# Autodesk Inventor assembly: Gearboxes_DesignTraining_Exercise1
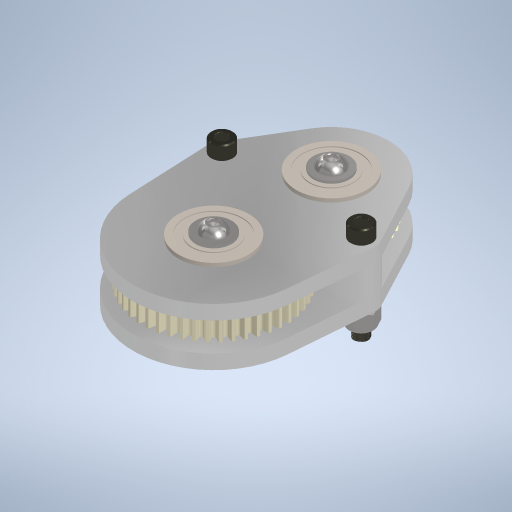
[picture p0: Inventor's stored thumbnail of the model, 512x512]
Saved by Autodesk Inventor 2024 (Build 280153000, 153)
## iProperties
Created: 2024-07-22
Part Number: Gearboxes_DesignTraining_Exercise1
Document SubType Name: Assembly
Designer: Danielle
Author: Danielle
## Documents named in this file (12)
- C:\Users\micha\OneDrive\Documents\GitHub\1622-2024-Assignments\Danielle\Gearboxes_DesignTraining_Exercise1.iam
- C:\Users\micha\OneDrive\Documents\BottomPlate.ipt
- C:\Users\micha\OneDrive\Documents\TopPlate.ipt
- C:\Users\micha\Downloads\WCP-0707 (1)\WCP-0707 (1).ipt
- C:\Users\micha\Downloads\WCP-0188 (1)\WCP-0188 (1).ipt
- C:\Users\micha\Downloads\WCP-0783 (1)\WCP-0783 (1).ipt
- C:\Users\micha\Downloads\WCP-0783\0.5 in long x 0.5 in wide x 0.257 in tap standoff.ipt
- C:\Users\micha\OneDrive\Documents\1.123 in. Hex Shaft.ipt
- C:\Users\micha\Downloads\92949A535_18-8 Stainless Steel Button Head Hex Drive Screw\92949A535_18-8 Stainless Steel Button Head Hex Drive Screw.ipt
- C:\Users\micha\Downloads\90107A029_316 Stainless Steel Washer\90107A029_316 Stainless Steel Washer.ipt
- C:\Users\micha\OneDrive\Documents\GitHub\1622-2024-Assignments\COTS Library\Fasteners\Bolts\Socket-Head\0.25-20\COTS_90044A123_Black-Oxide Alloy Steel Socket Head Screw.ipt
- C:\Users\micha\Downloads\97135A414_High-Strength Steel Nylon-Insert Locknut (1)\97135A414_High-Strength Steel Nylon-Insert Locknut (1).ipt
## Components (24 placed, 11 different names)
1. BottomPlate:1 — Mate:1, Mate:2, Mate:3, Mate:4, Mate:5, Mate:6, Mate:7, Mate:8, Mate:13, Mate:14, Mate:15, Mate:16, Mate:17, Mate:18, Mate:47, Mate:48
2. TopPlate:1 — Mate:1, Mate:2, Mate:3, Mate:4, Mate:9, Mate:10, Mate:11, Mate:12, Flush:5, Flush:6, Flush:7, Mate:41, Mate:42, Mate:43, Mate:44
3. WCP-0707 (1):1 — Mate:6, Flush:1, Flush:2, Angle:1, Angle:2
4. WCP-0188 (1):1 — Mate:5, Flush:1, Flush:2, Mate:19, Mate:20, Angle:3, Angle:4
5. WCP-0783 (1):1 — Mate:8, Mate:14, Angle:1, Mate:28
6. WCP-0783 (1):2 — Mate:10, Mate:11, Angle:2, Flush:9, Mate:22, Angle:5, Mate:26
7. WCP-0783 (1):3 — Mate:9, Mate:12, Mate:20, Angle:4, Mate:21, Flush:8, Angle:6, Mate:24
8. WCP-0783 (1):4 — Mate:7, Mate:13, Mate:19, Angle:3, Mate:29, Mate:30
9. 0.5 in long x 0.5 in wide x 0.257 in tap standoff:1 — Mate:15, Mate:16
10. 0.5 in long x 0.5 in wide x 0.257 in tap standoff:2 — Mate:17, Mate:18
11. 1.123 in. Hex Shaft:1 — Mate:21, Flush:8, Angle:6, Mate:23, Mate:31, Mate:33, Mate:35, Angle:8
12. 1.123 in. Hex Shaft:2 — Flush:9, Mate:22, Angle:5, Mate:25, Mate:27, Mate:32, Mate:34, Angle:7, Mate:36
13. 92949A535_18-8 Stainless Steel Button Head Hex Drive Screw:1 — Mate:33, Mate:39
14. 90107A029_316 Stainless Steel Washer:1 — Mate:23, Mate:24, Mate:35, Mate:39
15. 92949A535_18-8 Stainless Steel Button Head Hex Drive Screw:2 — Mate:32, Mate:37
16. 90107A029_316 Stainless Steel Washer:2 — Mate:29, Mate:30, Angle:8, Mate:38
17. 92949A535_18-8 Stainless Steel Button Head Hex Drive Screw:3 — Mate:31, Mate:38
18. 90107A029_316 Stainless Steel Washer:3 — Mate:25, Mate:26, Angle:7, Mate:40
19. 92949A535_18-8 Stainless Steel Button Head Hex Drive Screw:4 — Mate:34, Mate:40
20. 90107A029_316 Stainless Steel Washer:4 — Mate:27, Mate:28, Mate:36, Mate:37
21. COTS_90044A123_Black-Oxide Alloy Steel Socket Head Screw:1 — Mate:41, Mate:42, Mate:45
22. COTS_90044A123_Black-Oxide Alloy Steel Socket Head Screw:2 — Mate:43, Mate:44, Mate:46
23. 97135A414_High-Strength Steel Nylon-Insert Locknut (1):1 — Mate:45, Mate:47
24. 97135A414_High-Strength Steel Nylon-Insert Locknut (1):2 — Mate:46, Mate:48
## Relationships (63: Mate 48, Angle 8, Flush 7)
- Mate:1: BottomPlate:1 ↔ TopPlate:1
- Mate:2: BottomPlate:1 ↔ TopPlate:1
- Mate:3: BottomPlate:1 ↔ TopPlate:1
- Mate:4: BottomPlate:1 ↔ TopPlate:1
- Mate:5: BottomPlate:1 ↔ WCP-0188 (1):1
- Mate:6: BottomPlate:1 ↔ WCP-0707 (1):1
- Flush:1: WCP-0707 (1):1 ↔ WCP-0188 (1):1
- Mate:7: BottomPlate:1 ↔ WCP-0783 (1):4
- Mate:8: BottomPlate:1 ↔ WCP-0783 (1):1
- Mate:9: TopPlate:1 ↔ WCP-0783 (1):3
- Mate:10: TopPlate:1 ↔ WCP-0783 (1):2
- Mate:11: TopPlate:1 ↔ WCP-0783 (1):2
- Mate:12: TopPlate:1 ↔ WCP-0783 (1):3
- Mate:13: BottomPlate:1 ↔ WCP-0783 (1):4
- Mate:14: BottomPlate:1 ↔ WCP-0783 (1):1
- Mate:15: BottomPlate:1 ↔ 0.5 in long x 0.5 in wide x 0.257 in tap standoff:1
- Mate:16: BottomPlate:1 ↔ 0.5 in long x 0.5 in wide x 0.257 in tap standoff:1
- Mate:17: BottomPlate:1 ↔ 0.5 in long x 0.5 in wide x 0.257 in tap standoff:2
- Mate:18: BottomPlate:1 ↔ 0.5 in long x 0.5 in wide x 0.257 in tap standoff:2
- Flush:2: WCP-0707 (1):1 ↔ WCP-0188 (1):1
- Mate:19: WCP-0188 (1):1 ↔ WCP-0783 (1):4
- Mate:20: WCP-0188 (1):1 ↔ WCP-0783 (1):3
- Angle:1 (0 deg): WCP-0707 (1):1 ↔ WCP-0783 (1):1
- Angle:2 (0 deg): WCP-0707 (1):1 ↔ WCP-0783 (1):2
- Angle:3 (0 deg): WCP-0188 (1):1 ↔ WCP-0783 (1):4
- Angle:4 (0 deg): WCP-0188 (1):1 ↔ WCP-0783 (1):3
- Flush:5: TopPlate:1
- Flush:6: TopPlate:1
- Flush:7: TopPlate:1
- Mate:21: WCP-0783 (1):3 ↔ 1.123 in. Hex Shaft:1
- Flush:8: WCP-0783 (1):3 ↔ 1.123 in. Hex Shaft:1
- Flush:9: WCP-0783 (1):2 ↔ 1.123 in. Hex Shaft:2
- Mate:22: WCP-0783 (1):2 ↔ 1.123 in. Hex Shaft:2
- Angle:5 (0 deg): WCP-0783 (1):2 ↔ 1.123 in. Hex Shaft:2
- Angle:6 (0 deg): WCP-0783 (1):3 ↔ 1.123 in. Hex Shaft:1
- Mate:23: 1.123 in. Hex Shaft:1 ↔ 90107A029_316 Stainless Steel Washer:1
- Mate:24: WCP-0783 (1):3 ↔ 90107A029_316 Stainless Steel Washer:1
- Mate:25: 1.123 in. Hex Shaft:2 ↔ 90107A029_316 Stainless Steel Washer:3
- Mate:26: WCP-0783 (1):2 ↔ 90107A029_316 Stainless Steel Washer:3
- Mate:27: 1.123 in. Hex Shaft:2 ↔ 90107A029_316 Stainless Steel Washer:4
- Mate:28: WCP-0783 (1):1 ↔ 90107A029_316 Stainless Steel Washer:4
- Mate:29: WCP-0783 (1):4 ↔ 90107A029_316 Stainless Steel Washer:2
- Mate:30: WCP-0783 (1):4 ↔ 90107A029_316 Stainless Steel Washer:2
- Mate:31: 1.123 in. Hex Shaft:1 ↔ 92949A535_18-8 Stainless Steel Button Head Hex Drive Screw:3
- Mate:32: 1.123 in. Hex Shaft:2 ↔ 92949A535_18-8 Stainless Steel Button Head Hex Drive Screw:2
- Mate:33: 1.123 in. Hex Shaft:1 ↔ 92949A535_18-8 Stainless Steel Button Head Hex Drive Screw:1
- Mate:34: 1.123 in. Hex Shaft:2 ↔ 92949A535_18-8 Stainless Steel Button Head Hex Drive Screw:4
- Mate:35: 1.123 in. Hex Shaft:1 ↔ 90107A029_316 Stainless Steel Washer:1
- Angle:7 (0 deg): 1.123 in. Hex Shaft:2 ↔ 90107A029_316 Stainless Steel Washer:3
- Mate:36: 1.123 in. Hex Shaft:2 ↔ 90107A029_316 Stainless Steel Washer:4
- Angle:8 (0 deg): 1.123 in. Hex Shaft:1 ↔ 90107A029_316 Stainless Steel Washer:2
- Mate:37: 92949A535_18-8 Stainless Steel Button Head Hex Drive Screw:2 ↔ 90107A029_316 Stainless Steel Washer:4
- Mate:38: 90107A029_316 Stainless Steel Washer:2 ↔ 92949A535_18-8 Stainless Steel Button Head Hex Drive Screw:3
- Mate:39: 92949A535_18-8 Stainless Steel Button Head Hex Drive Screw:1 ↔ 90107A029_316 Stainless Steel Washer:1
- Mate:40: 90107A029_316 Stainless Steel Washer:3 ↔ 92949A535_18-8 Stainless Steel Button Head Hex Drive Screw:4
- Mate:41: TopPlate:1 ↔ COTS_90044A123_Black-Oxide Alloy Steel Socket Head Screw:1
- Mate:42: TopPlate:1 ↔ COTS_90044A123_Black-Oxide Alloy Steel Socket Head Screw:1
- Mate:43: TopPlate:1 ↔ COTS_90044A123_Black-Oxide Alloy Steel Socket Head Screw:2
- Mate:44: TopPlate:1 ↔ COTS_90044A123_Black-Oxide Alloy Steel Socket Head Screw:2
- Mate:45: COTS_90044A123_Black-Oxide Alloy Steel Socket Head Screw:1 ↔ 97135A414_High-Strength Steel Nylon-Insert Locknut (1):1
- Mate:46: COTS_90044A123_Black-Oxide Alloy Steel Socket Head Screw:2 ↔ 97135A414_High-Strength Steel Nylon-Insert Locknut (1):2
- Mate:47: BottomPlate:1 ↔ 97135A414_High-Strength Steel Nylon-Insert Locknut (1):1
- Mate:48: BottomPlate:1 ↔ 97135A414_High-Strength Steel Nylon-Insert Locknut (1):2
